# Autodesk Inventor assembly: flat 0.25v3
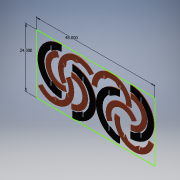
[picture p0: Inventor's stored thumbnail of the model, 180x180]
Saved by Autodesk Inventor 2016 (Build 200138000, 138)
## iProperties
Created: 2016-02-06
Part Number: flat 0.25v3
Document SubType Name: Assembly
Designer: Scott
Author: Scott
## Documents named in this file (4)
- F:\Dropbox\CubeSat\Cleaned_Up_Helmholtz_Model_for_Manual\Flat_Patterns\Flat_0.25.iam
- F:\Dropbox\CubeSat\Cleaned_Up_Helmholtz_Model_for_Manual\Parts\Small_Coil_Inner.ipt
- F:\Dropbox\CubeSat\Cleaned_Up_Helmholtz_Model_for_Manual\Parts\Medium_Coil_Inner.ipt
- F:\Dropbox\CubeSat\Cleaned_Up_Helmholtz_Model_for_Manual\Parts\Large_Coil_Inner.ipt
## Components (12 placed, 3 different names)
1. Small_Coil_Inner:1 — Flush:2
2. Medium_Coil_Inner:1 — Flush:1, Flush:2
3. Large_Coil_Inner:1 — Flush:1, Flush:10, Flush:11
4. Small_Coil_Inner:2 — Flush:3
5. Medium_Coil_Inner:2 — Flush:3, Flush:4
6. Large_Coil_Inner:2 — Flush:4, Flush:5, Flush:10
7. Small_Coil_Inner:3 — Flush:7
8. Medium_Coil_Inner:3 — Flush:6, Flush:7
9. Large_Coil_Inner:3 — Flush:5, Flush:6
10. Small_Coil_Inner:4 — Flush:12
11. Medium_Coil_Inner:4 — Flush:8, Flush:12
12. Large_Coil_Inner:4 — Flush:8, Flush:11
## Relationships (11: Flush 11)
- Flush:1: Medium_Coil_Inner:1 ↔ Large_Coil_Inner:1
- Flush:2: Small_Coil_Inner:1 ↔ Medium_Coil_Inner:1
- Flush:3: Small_Coil_Inner:2 ↔ Medium_Coil_Inner:2
- Flush:4: Medium_Coil_Inner:2 ↔ Large_Coil_Inner:2
- Flush:5: Large_Coil_Inner:2 ↔ Large_Coil_Inner:3
- Flush:6: Medium_Coil_Inner:3 ↔ Large_Coil_Inner:3
- Flush:7: Small_Coil_Inner:3 ↔ Medium_Coil_Inner:3
- Flush:8: Medium_Coil_Inner:4 ↔ Large_Coil_Inner:4
- Flush:10: Large_Coil_Inner:1 ↔ Large_Coil_Inner:2
- Flush:11: Large_Coil_Inner:1 ↔ Large_Coil_Inner:4
- Flush:12: Small_Coil_Inner:4 ↔ Medium_Coil_Inner:4
